# Autodesk Inventor assembly: tmp
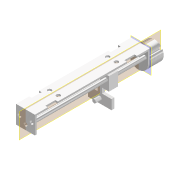
[picture p0: Inventor's stored thumbnail of the model, 180x180]
Saved by Autodesk Inventor 2022 (Build 260153000, 153)
## iProperties
Created: 2022-05-21
Part Number: tmp
Document SubType Name: Assembly
Designer: diederichbenedict
Author: diederichbenedict
## Documents named in this file (3)
- C:\Users\diederichbenedict\Dropbox\Dokumente\Promotion\PROJECTS\TIRFImager\INVENTOR\tmp.iam
- C:\Users\diederichbenedict\Dropbox\Dokumente\Promotion\PROJECTS\TIRFImager\INVENTOR\30_Cube_Insert_Filter_Revolver_Filter_base_triple_linearmotor.ipt
- C:\Users\diederichbenedict\Dropbox\Dokumente\Promotion\PROJECTS\TIRFImager\INVENTOR\Assebmly_Linear_Stepper_90mm.iam
## Components (2 placed, 2 different names)
1. 30_Cube_Insert_Filter_Revolver_Filter_base_triple_linearmotor:1
2. Assebmly_Linear_Stepper_90mm:1 [sub-assembly]
## Relationships (3: Mate 3)
- [Mate] (0.5 mm): 30_Cube_Insert_Filter_Revolver_Filter_base_triple_linearmotor:1 ↔ Assebmly_Linear_Stepper_90mm:1
- [Mate] (0.5 mm): 30_Cube_Insert_Filter_Revolver_Filter_base_triple_linearmotor:1 ↔ Assebmly_Linear_Stepper_90mm:1
- [Mate]: 30_Cube_Insert_Filter_Revolver_Filter_base_triple_linearmotor:1 ↔ Assebmly_Linear_Stepper_90mm:1
